# Autodesk Inventor assembly: 回転アームテスト
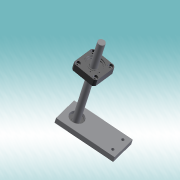
[picture p0: Inventor's stored thumbnail of the model, 180x180]
Saved by Autodesk Inventor 2015 (Build 190159000, 159)
## iProperties
Created: 2016-03-21
Part Number: 回転アームテスト
Document SubType Name: 溶接アセンブリ
Designer: buzztaka
Weld Material: アルミニウム 6061、溶接
Mass: 82.3328 g
Surface Area: 315.874 cm^2
Volume: 82.3328 cm^3
Density: 1 g/cm^3
Author: buzztaka
## Documents named in this file (5)
- C:\Users\buzztaka\Documents\tukuba\i-cart-middle_3d-model\計測輪アセンブル\回転アームテスト - コピー.iam
- C:\Users\buzztaka\Documents\tukuba\i-cart-middle_3d-model\計測輪アセンブル\回転軸取り付け板.ipt
- C:\Users\buzztaka\Documents\tukuba\i-cart-middle_3d-model\計測輪アセンブル\C-SFL6901ZZ.ipt
- C:\Users\buzztaka\Documents\tukuba\i-cart-middle_3d-model\計測輪アセンブル\回転軸.ipt
- C:\Users\buzztaka\Documents\tukuba\i-cart-middle_3d-model\計測輪アセンブル\ベアリングホルダ\BGSRB6201ZZ.iam
## Components (4 placed, 4 different names)
1. 回転軸取り付け板:2
2. C-SFL6901ZZ:2 — 挿入:3
3. 回転軸:1 — 挿入:3, 挿入:4
4. BGSRB6201ZZ:1 [sub-assembly] — 挿入:4
## Relationships (3: Insert 3)
- [Insert]: 回転軸取り付け板:2 ↔ C-SFL6901ZZ:2
- 挿入:3 [Insert] (10 mm): C-SFL6901ZZ:2 ↔ 回転軸:1
- 挿入:4 [Insert] (-60 mm): 回転軸:1 ↔ BGSRB6201ZZ:1
## Named parameters: d1_d0 = 0 mm
